# Autodesk Inventor assembly: espalda
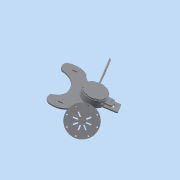
[picture p0: Inventor's stored thumbnail of the model, 180x180]
Saved by Autodesk Inventor 2015 (Build 190159000, 159)
## iProperties
Created: 2017-10-02
Part Number: espalda
Document SubType Name: Assembly
Designer: macbook
Author: macbook
## Documents named in this file (7)
- \\Mac\Home\Dropbox\cosplay\espalda\espalda.iam
- \\Mac\Home\Dropbox\cosplay\espalda\central.ipt
- \\Mac\Home\Dropbox\cosplay\espalda\centralmedio.ipt
- \\Mac\Home\Dropbox\cosplay\espalda\tapa.ipt
- \\Mac\Home\Dropbox\cosplay\espalda\base.ipt
- \\Mac\Home\Dropbox\cosplay\espalda\lados\brazo.ipt
- \\Mac\Home\Dropbox\cosplay\espalda\lados\base.ipt
## Components (9 placed, 5 different names)
1. central:1 — Rigid:1, Rigid:3
2. central:2 — Rigid:1, Rotational:2
3. central:3 — Rigid:4
4. central:4 — Rotational:1
5. centralmedio:1 — Rigid:3, Rigid:4
6. tapa:1 — Rotational:1
7. base:1 — Rotational:2, Mate:1, Mate:2, Mate:3
8. brazo:1 — Mate:1, Mate:2, Mate:3, Mate:4, Mate:5, Mate:6
9. base:2 — Mate:4, Mate:5, Mate:6
## Relationships (12: Mate 6, WeldJoint 4, RevoluteJoint 2)
- Rigid:1 [WeldJoint]: central:1 ↔ central:2
- [WeldJoint]: central:3 ↔ central:4
- Rigid:3 [WeldJoint]: central:1 ↔ centralmedio:1
- Rigid:4 [WeldJoint]: central:3 ↔ centralmedio:1
- Rotational:1 [RevoluteJoint]: central:4 ↔ tapa:1
- Rotational:2 [RevoluteJoint]: central:2 ↔ base:1
- Mate:1: base:1 ↔ brazo:1
- Mate:2: base:1 ↔ brazo:1
- Mate:3: base:1 ↔ brazo:1
- Mate:4: brazo:1 ↔ base:2
- Mate:5: brazo:1 ↔ base:2
- Mate:6: brazo:1 ↔ base:2
## Named parameters: d1_d0 = 0 mm
